# Autodesk Inventor assembly: Gearbox with neverest_MIR1
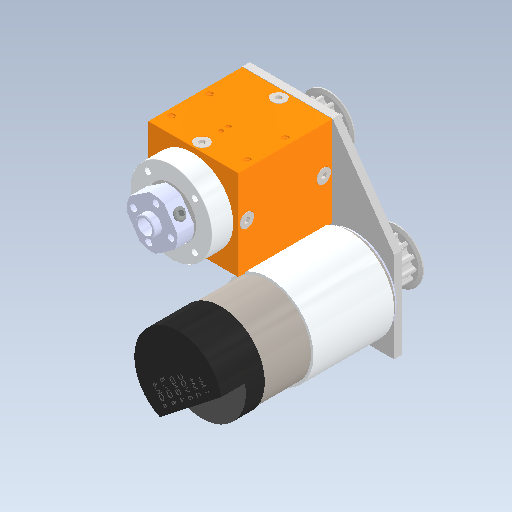
[picture p0: Inventor's stored thumbnail of the model, 512x512]
Saved by Autodesk Inventor 2020.2 (Build 242310000, 310)
## iProperties
Created: 2020-02-27
Part Number: Gearbox with neverest_MIR1
Document SubType Name: Assembly
Designer: deli
Author: deli
## Documents named in this file (8)
- C:\Users\deli\OneDrive - Eastside Preparatory School\FTC\Chassi\Gearbox with neverest_MIR1.iam
- C:\Users\deli\OneDrive - Eastside Preparatory School\FTC\Chassi\20-1 gearbox_MIR1.iam
- C:\Users\deli\OneDrive - Eastside Preparatory School\FTC\Chassi\.5 flanged bearing_MIR1.ipt
- C:\Users\deli\OneDrive - Eastside Preparatory School\FTC\Chassi\Motor and gearbox panel_MIR1.ipt
- C:\Users\deli\OneDrive - Eastside Preparatory School\FTC\Chassi\neveRest with 15T pinion_MIR1.iam
- C:\Users\deli\OneDrive - Eastside Preparatory School\FTC\Chassi\12T Pulley for neverest_MIR1.ipt
- C:\Users\deli\OneDrive - Eastside Preparatory School\FTC\Chassi\12T Pulley for gearbox_MIR1.ipt
- C:\Users\deli\OneDrive - Eastside Preparatory School\FTC\Chassi\Gearbox with neverest\Design Accelerator\Bevel Gears1_MIR1.iam
## Components (7 placed, 7 different names)
1. 20-1 gearbox_MIR1:1 [sub-assembly] — Mate:2, Mate:1, Flush:2, Mate:14, Angle:1
2. .5 flanged bearing_MIR1:1 — Mate:2, Mate:1
3. Motor and gearbox panel_MIR1:1
4. neveRest with 15T pinion_MIR1:1 [sub-assembly] — Mate:12, Mate:11, Flush:1
5. 12T Pulley for neverest_MIR1:1 — Mate:12, Mate:11, Flush:1
6. 12T Pulley for gearbox_MIR1:1 — Flush:2, Mate:14, Angle:1
7. Bevel Gears1_MIR1:1 [sub-assembly]
## Relationships (8: Mate 5, Flush 2, Angle 1)
- Mate:2: 20-1 gearbox_MIR1:1 ↔ .5 flanged bearing_MIR1:1
- Mate:1: 20-1 gearbox_MIR1:1 ↔ .5 flanged bearing_MIR1:1
- Mate:12: neveRest with 15T pinion_MIR1:1 ↔ 12T Pulley for neverest_MIR1:1
- Mate:11: neveRest with 15T pinion_MIR1:1 ↔ 12T Pulley for neverest_MIR1:1
- Flush:1: neveRest with 15T pinion_MIR1:1 ↔ 12T Pulley for neverest_MIR1:1
- Flush:2: 20-1 gearbox_MIR1:1 ↔ 12T Pulley for gearbox_MIR1:1
- Mate:14: 20-1 gearbox_MIR1:1 ↔ 12T Pulley for gearbox_MIR1:1
- Angle:1 (0 deg): 20-1 gearbox_MIR1:1 ↔ 12T Pulley for gearbox_MIR1:1
